# Autodesk Inventor assembly: SideChestPanel
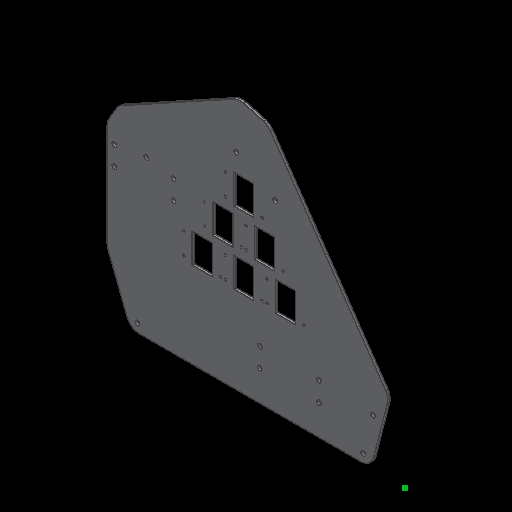
[picture p0: Inventor's stored thumbnail of the model, 512x512]
Saved by Autodesk Inventor 2025.2 (Build 292293000, 293)
## iProperties
Created: 2025-12-14
Part Number: SideChestPanel
Document SubType Name: Assembly
Designer: valer
Author: valer
## Documents named in this file (2)
- C:\Users\valer\Desktop\str1ker\cad\SideChestPanel.iam
- C:\Users\valer\Desktop\str1ker\cad\SideChestPanel.ipt
## Components (1 placed, 1 different names)
1. SideChestPanel:1 — Flush:3, Flush:4
## Relationships (2: Flush 2)
- Flush:3: SideChestPanel:1
- Flush:4: SideChestPanel:1
